# Autodesk Inventor assembly: M5 Screw with Tee Nut Reverse
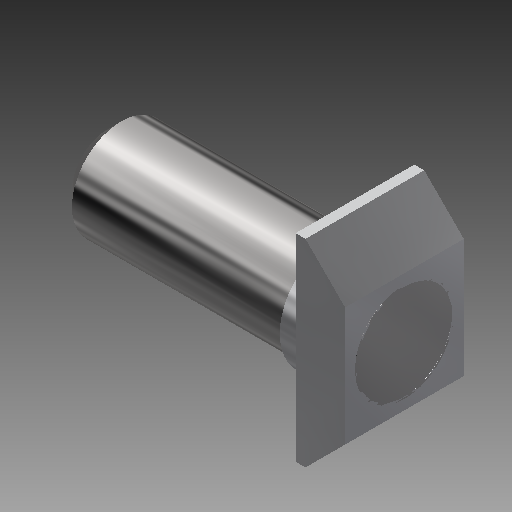
[picture p0: Inventor's stored thumbnail of the model, 512x512]
Saved by Autodesk Inventor 2017 (Build 210142000, 142)
## iProperties
Created: 2014-02-18
Part Number: M5 Screw with Tee Nut Reverse
Document SubType Name: Assembly
Designer: umr
Mass: 2.37189 g
Surface Area: 4.79898 cm^2
Volume: 0.378301 cm^3
Density: 6.26986 g/cm^3
Sending System: SolidWorks 2014
Last Author: Rory
Last Saved: 2016-05-20
Author: umr
## Documents named in this file (3)
- D:\SeniorProject\Models2\Gantry\Tee Nut With headless screw.iam
- D:\SeniorProject\Models2\Gantry\Tee Nut.ipt
- D:\SeniorProject\Models2\Gantry\M5ScrewWithoutNot.ipt
## Components (2 placed, 2 different names)
1. Tee Nut:1 — Mate:1, Flush:1
2. M5ScrewWithoutNot:1 — Mate:1, Flush:1
## Relationships (2: Mate 1, Flush 1)
- Mate:1: Tee Nut:1 ↔ M5ScrewWithoutNot:1
- Flush:1: Tee Nut:1 ↔ M5ScrewWithoutNot:1
